# Autodesk Inventor assembly: Integrated Assembly Attempt
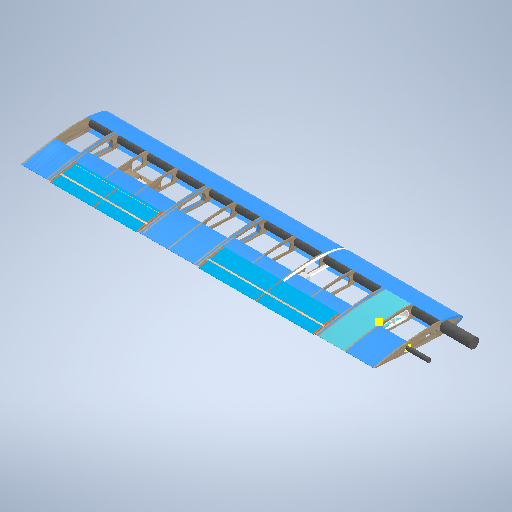
[picture p0: Inventor's stored thumbnail of the model, 512x512]
Saved by Autodesk Inventor 2025.1 (Build 291241000, 241)
## iProperties
Created: 2025-02-02
Part Number: Integrated Assembly Attempt
Document SubType Name: Assembly
Designer: Imist
Author: Imist
## Documents named in this file (39)
- C:\Users\hjbre\OneDrive - University of Bristol\CAD Files\Full Assembly\P Wing\Integrated Assembly P Wing.iam
- C:\Users\hjbre\OneDrive - University of Bristol\CAD Files\Full Assembly\P Wing\1P.02.01.01-HB-FalseRearSpar.ipt
- C:\Users\hjbre\OneDrive - University of Bristol\CAD Files\Full Assembly\P Wing\1P.02.01.02-RN-MainSpar.ipt
- C:\Users\hjbre\OneDrive - University of Bristol\CAD Files\Full Assembly\P Wing\1P.01.01.13-HB-Rib13.ipt
- C:\Users\hjbre\OneDrive - University of Bristol\CAD Files\Full Assembly\P Wing\1P.01.02.03-HB-TrailingEdgeTipEnd.ipt
- C:\Users\hjbre\OneDrive - University of Bristol\CAD Files\Full Assembly\P Wing\1P.01.01.12-HB-Rib12.ipt
- C:\Users\hjbre\OneDrive - University of Bristol\CAD Files\Full Assembly\P Wing\1P.01.04.04-HB-Rib12Foam.ipt
- C:\Users\hjbre\OneDrive - University of Bristol\CAD Files\Full Assembly\P Wing\1P.01.03.04-HB-AileronFoamOuter.ipt
- C:\Users\hjbre\OneDrive - University of Bristol\CAD Files\Full Assembly\P Wing\1P.01.01.11-HB-Rib11.ipt
- C:\Users\hjbre\OneDrive - University of Bristol\CAD Files\Full Assembly\P Wing\1P.01.03.05-HB-AileronFoamInner.ipt
- C:\Users\hjbre\OneDrive - University of Bristol\CAD Files\Full Assembly\P Wing\1P.01.01.10-HB-Rib10a.ipt
- C:\Users\hjbre\OneDrive - University of Bristol\CAD Files\Full Assembly\P Wing\1P.01.01.09-HB-Rib9.ipt
- C:\Users\hjbre\OneDrive - University of Bristol\CAD Files\Full Assembly\P Wing\1P.01.04.03-HB-Rib9Foam.ipt
- C:\Users\hjbre\OneDrive - University of Bristol\CAD Files\Full Assembly\P Wing\1P.01.02.02-HB-TrailingEdgeSand-Rib.ipt
- C:\Users\hjbre\OneDrive - University of Bristol\CAD Files\Full Assembly\P Wing\1P.01.01.08-HB-Rib8.ipt
- C:\Users\hjbre\OneDrive - University of Bristol\CAD Files\Full Assembly\P Wing\1P.01.01.07-HB-Rib7.ipt
- C:\Users\hjbre\OneDrive - University of Bristol\CAD Files\Full Assembly\P Wing\1P.01.04.02-HB-Rib7Foam.ipt
- C:\Users\hjbre\OneDrive - University of Bristol\CAD Files\Full Assembly\P Wing\1P.01.03.01-HB-FlapFoamOuter.ipt
- C:\Users\hjbre\OneDrive - University of Bristol\CAD Files\Full Assembly\P Wing\1P.01.01.06-HB-Rib6.ipt
- C:\Users\hjbre\OneDrive - University of Bristol\CAD Files\Full Assembly\P Wing\1P.01.03.03-HB-FlapFoam.ipt
- C:\Users\hjbre\OneDrive - University of Bristol\CAD Files\Full Assembly\P Wing\1P.01.01.05-HB-Rib5.ipt
- C:\Users\hjbre\OneDrive - University of Bristol\CAD Files\Full Assembly\P Wing\1P.01.05.01-HB-PressureTap.ipt
- C:\Users\hjbre\OneDrive - University of Bristol\CAD Files\Full Assembly\P Wing\1P.01.03.02-HB-FlapFoamPressTap.ipt
- C:\Users\hjbre\OneDrive - University of Bristol\CAD Files\Full Assembly\P Wing\1P.01.01.04-HB-Rib4.ipt
- C:\Users\hjbre\OneDrive - University of Bristol\CAD Files\Full Assembly\P Wing\1P.01.01.03-HB-Rib3.ipt
- C:\Users\hjbre\OneDrive - University of Bristol\CAD Files\Full Assembly\P Wing\1P.01.04.01-HB-Rib3Foam.ipt
- C:\Users\hjbre\OneDrive - University of Bristol\CAD Files\Full Assembly\P Wing\1P.01.02.06-HB-Trailing adge access panel.ipt
- C:\Users\hjbre\OneDrive - University of Bristol\CAD Files\Full Assembly\P Wing\1P.01.01.02-HB-Rib2.ipt
- C:\Users\hjbre\OneDrive - University of Bristol\CAD Files\Full Assembly\P Wing\1P.01.02.01-HB-TrailingEdgeRootEnd.ipt
- C:\Users\hjbre\OneDrive - University of Bristol\CAD Files\Full Assembly\P Wing\1P.01.01.01-HB-Rib1.ipt
- C:\Users\hjbre\OneDrive - University of Bristol\CAD Files\Full Assembly\P Wing\1P.01.05.03-HB-PlatformFinal.ipt
- C:\Users\hjbre\OneDrive - University of Bristol\CAD Files\Full Assembly\P Wing\2P.03.01.02.JW.AilSerCage.ipt
- C:\Users\hjbre\OneDrive - University of Bristol\CAD Files\Full Assembly\P Wing\1P.01.02.05-HB-LeadingEdgeTipEnd.ipt
- C:\Users\hjbre\OneDrive - University of Bristol\CAD Files\Full Assembly\P Wing\1P.01.02.04-HB-LeadingEdgeRootEnd.ipt
- C:\Users\hjbre\OneDrive - University of Bristol\CAD Files\Full Assembly\P Wing\AilServoRep (1).ipt
- C:\Users\hjbre\OneDrive - University of Bristol\CAD Files\Full Assembly\P Wing\servoRep (1).ipt
- C:\Users\hjbre\OneDrive - University of Bristol\CAD Files\Full Assembly\P Wing\2A.01.01.01.IM.FlapAssembly.iam
- C:\Users\hjbre\OneDrive - University of Bristol\CAD Files\Full Assembly\P Wing\2P.03.01.00.05.IM.Bearing8x12x3.5.ipt
- C:\Users\hjbre\OneDrive - University of Bristol\CAD Files\Full Assembly\P Wing\2A.01.01.02.IM.AileronAssembly.iam
## Components (48 placed, 38 different names)
1. 1P.02.01.01-HB-FalseRearSpar:1 — Mate:5, Mate:6, Mate:7, Mate:8, Mate:10, Rotational:2, Rigid:6, Rigid:8, Rigid:23
2. 1P.02.01.02-RN-MainSpar:1 — Mate:1, Mate:2, Mate:3, Mate:4, Mate:9, Mate:11, Rotational:1
3. 1P.01.01.13-HB-Rib13:1 — Rotational:1, Rotational:2, Rigid:1, Rigid:2, Rigid:3, Rigid:4, Rigid:5, Rigid:9, Rigid:10, Rigid:17, Rigid:19, Rigid:21, Rigid:24, Rigid:25, Rigid:26, Rigid:28, Rigid:30
4. 1P.01.02.03-HB-TrailingEdgeTipEnd:2 — Rigid:1
5. 1P.01.01.12-HB-Rib12:1 — Rigid:2
6. 1P.01.04.04-HB-Rib12Foam:1 — Rigid:3
7. 1P.01.01.12-HB-Rib12:2 — Rigid:4, Rotational:3, Rigid:35
8. 1P.01.03.04-HB-AileronFoamOuter:1 — Rotational:3, Rotational:4
9. 1P.01.01.11-HB-Rib11:1 — Rigid:5
10. 1P.01.03.04-HB-AileronFoamOuter:2 — Rigid:7
11. 1P.01.03.05-HB-AileronFoamInner:1 — Rotational:4, Rigid:7
12. 1P.01.01.10-HB-Rib10a:1 — Rigid:6, Rigid:29
13. 1P.01.01.09-HB-Rib9:1 — Rigid:8, Rigid:36
14. 1P.01.04.03-HB-Rib9Foam:1 — Rigid:9
15. 1P.01.01.09-HB-Rib9:2 — Rigid:10, Rigid:11
16. 1P.01.02.02-HB-TrailingEdgeSand-Rib:1 — Rigid:11, Rigid:12
17. 1P.01.01.08-HB-Rib8:1 — Rigid:12, Rigid:13
18. 1P.01.02.02-HB-TrailingEdgeSand-Rib:2 — Rigid:13, Rigid:14
19. 1P.01.01.07-HB-Rib7:1 — Rigid:14, Rigid:15
20. 1P.01.04.02-HB-Rib7Foam:1 — Rigid:15, Rigid:16
21. 1P.01.01.07-HB-Rib7:2 — Rigid:16, Rotational:5, Rigid:33
22. 1P.01.03.01-HB-FlapFoamOuter:1 — Rotational:5, Rigid:18
23. 1P.01.01.06-HB-Rib6:1 — Rigid:17
24. 1P.01.03.03-HB-FlapFoam:1 — Rigid:18, Rotational:6, Rigid:20
25. 1P.01.01.05-HB-Rib5:1 — Rigid:19, Slider:1
26. 1P.01.05.01-HB-PressureTap:1 — Rotational:6
27. 1P.01.03.02-HB-FlapFoamPressTap:1 — Rigid:20, Rigid:22
28. 1P.01.01.04-HB-Rib4:1 — Rigid:21
29. 1P.01.03.01-HB-FlapFoamOuter:2 — Rigid:22
30. 1P.01.01.03-HB-Rib3:1 — Rigid:25, Rotational:7
31. 1P.01.01.03-HB-Rib3:2 — Rigid:23, Rigid:34
32. 1P.01.04.01-HB-Rib3Foam:1 — Rigid:24
33. 1P.01.02.06-HB-Trailing adge access panel:1 — Rotational:7
34. 1P.01.01.02-HB-Rib2:1 — Rigid:26, Rigid:27, Rotational:8
35. 1P.01.02.01-HB-TrailingEdgeRootEnd:1 — Rigid:27
36. 1P.01.01.01-HB-Rib1:1 — Rigid:28, Rigid:31
37. 1P.01.05.03-HB-PlatformFinal:1 — Rotational:8
38. 2P.03.01.02.JW.AilSerCage:1 — Rigid:29, Rigid:32
39. 1P.01.02.05-HB-LeadingEdgeTipEnd:1 — Rigid:30
40. 1P.01.02.04-HB-LeadingEdgeRootEnd:1 — Rigid:31
41. AilServoRep (1):1 — Rigid:32
42. servoRep (1):1 — Slider:1
43. 2A.01.01.01.IM.FlapAssembly:1 [sub-assembly] — Rotational:9
44. 2P.03.01.00.05.IM.Bearing8x12x3.5:1 — Rigid:33
45. 2P.03.01.00.05.IM.Bearing8x12x3.5:2 — Rigid:34, Rotational:9
46. 2P.03.01.00.05.IM.Bearing8x12x3.5:3 — Rigid:35, Rotational:10
47. 2P.03.01.00.05.IM.Bearing8x12x3.5:4 — Rigid:36
48. 2A.01.01.02.IM.AileronAssembly:1 [sub-assembly] — Rotational:10
## Relationships (58: WeldJoint 36, Mate 11, RevoluteJoint 10, TranslationJoint 1)
- Mate:1: 1P.02.01.02-RN-MainSpar:1
- Mate:2: 1P.02.01.02-RN-MainSpar:1
- Mate:3: 1P.02.01.02-RN-MainSpar:1
- Mate:4: 1P.02.01.02-RN-MainSpar:1
- Mate:5 (126.581 mm): 1P.02.01.01-HB-FalseRearSpar:1
- Mate:6 (126.026 mm): 1P.02.01.01-HB-FalseRearSpar:1
- Mate:7: 1P.02.01.01-HB-FalseRearSpar:1
- Mate:8: 1P.02.01.01-HB-FalseRearSpar:1
- Mate:9: 1P.02.01.02-RN-MainSpar:1
- Mate:10: 1P.02.01.01-HB-FalseRearSpar:1
- Mate:11 (1300 mm): 1P.02.01.02-RN-MainSpar:1
- Rotational:1 [RevoluteJoint]: 1P.02.01.02-RN-MainSpar:1 ↔ 1P.01.01.13-HB-Rib13:1
- Rotational:2 [RevoluteJoint]: 1P.02.01.01-HB-FalseRearSpar:1 ↔ 1P.01.01.13-HB-Rib13:1
- Rigid:1 [WeldJoint] (-4 mm): 1P.01.01.13-HB-Rib13:1 ↔ 1P.01.02.03-HB-TrailingEdgeTipEnd:2
- Rigid:2 [WeldJoint] (-87 mm): 1P.01.01.13-HB-Rib13:1 ↔ 1P.01.01.12-HB-Rib12:1
- Rigid:3 [WeldJoint] (-91 mm): 1P.01.01.13-HB-Rib13:1 ↔ 1P.01.04.04-HB-Rib12Foam:1
- Rigid:4 [WeldJoint] (-96 mm): 1P.01.01.13-HB-Rib13:1 ↔ 1P.01.01.12-HB-Rib12:2
- Rotational:3 [RevoluteJoint]: 1P.01.01.12-HB-Rib12:2 ↔ 1P.01.03.04-HB-AileronFoamOuter:1
- Rigid:5 [WeldJoint] (-198 mm): 1P.01.01.13-HB-Rib13:1 ↔ 1P.01.01.11-HB-Rib11:1
- Rotational:4 [RevoluteJoint] (4 mm): 1P.01.03.04-HB-AileronFoamOuter:1 ↔ 1P.01.03.05-HB-AileronFoamInner:1
- Rigid:6 [WeldJoint] (-298 mm): 1P.02.01.01-HB-FalseRearSpar:1 ↔ 1P.01.01.10-HB-Rib10a:1
- Rigid:7 [WeldJoint] (4 mm): 1P.01.03.04-HB-AileronFoamOuter:2 ↔ 1P.01.03.05-HB-AileronFoamInner:1
- Rigid:8 [WeldJoint] (-400 mm): 1P.02.01.01-HB-FalseRearSpar:1 ↔ 1P.01.01.09-HB-Rib9:1
- Rigid:9 [WeldJoint] (-404 mm): 1P.01.01.13-HB-Rib13:1 ↔ 1P.01.04.03-HB-Rib9Foam:1
- Rigid:10 [WeldJoint] (-409 mm): 1P.01.01.13-HB-Rib13:1 ↔ 1P.01.01.09-HB-Rib9:2
- Rigid:11 [WeldJoint]: 1P.01.01.09-HB-Rib9:2 ↔ 1P.01.02.02-HB-TrailingEdgeSand-Rib:1
- Rigid:12 [WeldJoint]: 1P.01.02.02-HB-TrailingEdgeSand-Rib:1 ↔ 1P.01.01.08-HB-Rib8:1
- Rigid:13 [WeldJoint]: 1P.01.01.08-HB-Rib8:1 ↔ 1P.01.02.02-HB-TrailingEdgeSand-Rib:2
- Rigid:14 [WeldJoint]: 1P.01.02.02-HB-TrailingEdgeSand-Rib:2 ↔ 1P.01.01.07-HB-Rib7:1
- Rigid:15 [WeldJoint]: 1P.01.01.07-HB-Rib7:1 ↔ 1P.01.04.02-HB-Rib7Foam:1
- Rigid:16 [WeldJoint]: 1P.01.04.02-HB-Rib7Foam:1 ↔ 1P.01.01.07-HB-Rib7:2
- Rotational:5 [RevoluteJoint]: 1P.01.01.07-HB-Rib7:2 ↔ 1P.01.03.01-HB-FlapFoamOuter:1
- Rigid:17 [WeldJoint] (-698 mm): 1P.01.01.13-HB-Rib13:1 ↔ 1P.01.01.06-HB-Rib6:1
- Rigid:18 [WeldJoint] (4 mm): 1P.01.03.01-HB-FlapFoamOuter:1 ↔ 1P.01.03.03-HB-FlapFoam:1
- Rigid:19 [WeldJoint] (-798 mm): 1P.01.01.13-HB-Rib13:1 ↔ 1P.01.01.05-HB-Rib5:1
- Rotational:6 [RevoluteJoint] (4 mm): 1P.01.03.03-HB-FlapFoam:1 ↔ 1P.01.05.01-HB-PressureTap:1
- Rigid:20 [WeldJoint] (12 mm): 1P.01.03.03-HB-FlapFoam:1 ↔ 1P.01.03.02-HB-FlapFoamPressTap:1
- Rigid:21 [WeldJoint] (-898 mm): 1P.01.01.13-HB-Rib13:1 ↔ 1P.01.01.04-HB-Rib4:1
- Rigid:22 [WeldJoint] (4 mm): 1P.01.03.02-HB-FlapFoamPressTap:1 ↔ 1P.01.03.01-HB-FlapFoamOuter:2
- Rigid:23 [WeldJoint] (-1000 mm): 1P.02.01.01-HB-FalseRearSpar:1 ↔ 1P.01.01.03-HB-Rib3:2
- Rigid:24 [WeldJoint] (-1004 mm): 1P.01.01.13-HB-Rib13:1 ↔ 1P.01.04.01-HB-Rib3Foam:1
- Rigid:25 [WeldJoint] (-1009 mm): 1P.01.01.13-HB-Rib13:1 ↔ 1P.01.01.03-HB-Rib3:1
- Rotational:7 [RevoluteJoint]: 1P.01.01.03-HB-Rib3:1 ↔ 1P.01.02.06-HB-Trailing adge access panel:1
- Rigid:26 [WeldJoint] (-1098 mm): 1P.01.01.13-HB-Rib13:1 ↔ 1P.01.01.02-HB-Rib2:1
- Rigid:27 [WeldJoint]: 1P.01.01.02-HB-Rib2:1 ↔ 1P.01.02.01-HB-TrailingEdgeRootEnd:1
- Rigid:28 [WeldJoint] (-1196 mm): 1P.01.01.13-HB-Rib13:1 ↔ 1P.01.01.01-HB-Rib1:1
- Rotational:8 [RevoluteJoint]: 1P.01.01.02-HB-Rib2:1 ↔ 1P.01.05.03-HB-PlatformFinal:1
- Rigid:29 [WeldJoint]: 1P.01.01.10-HB-Rib10a:1 ↔ 2P.03.01.02.JW.AilSerCage:1
- Rigid:30 [WeldJoint]: 1P.01.01.13-HB-Rib13:1 ↔ 1P.01.02.05-HB-LeadingEdgeTipEnd:1
- Rigid:31 [WeldJoint]: 1P.01.01.01-HB-Rib1:1 ↔ 1P.01.02.04-HB-LeadingEdgeRootEnd:1
- Rigid:32 [WeldJoint]: 2P.03.01.02.JW.AilSerCage:1 ↔ AilServoRep (1):1
- Slider:1 [TranslationJoint]: 1P.01.01.05-HB-Rib5:1 ↔ servoRep (1):1
- Rigid:33 [WeldJoint]: 1P.01.01.07-HB-Rib7:2 ↔ 2P.03.01.00.05.IM.Bearing8x12x3.5:1
- Rigid:34 [WeldJoint]: 1P.01.01.03-HB-Rib3:2 ↔ 2P.03.01.00.05.IM.Bearing8x12x3.5:2
- Rotational:9 [RevoluteJoint] (-1 mm): 2A.01.01.01.IM.FlapAssembly:1 ↔ 2P.03.01.00.05.IM.Bearing8x12x3.5:2
- Rigid:35 [WeldJoint]: 1P.01.01.12-HB-Rib12:2 ↔ 2P.03.01.00.05.IM.Bearing8x12x3.5:3
- Rigid:36 [WeldJoint]: 1P.01.01.09-HB-Rib9:1 ↔ 2P.03.01.00.05.IM.Bearing8x12x3.5:4
- Rotational:10 [RevoluteJoint] (-1 mm): 2P.03.01.00.05.IM.Bearing8x12x3.5:3 ↔ 2A.01.01.02.IM.AileronAssembly:1
